# Autodesk Inventor assembly: Atom_3_Lite_Upgrade
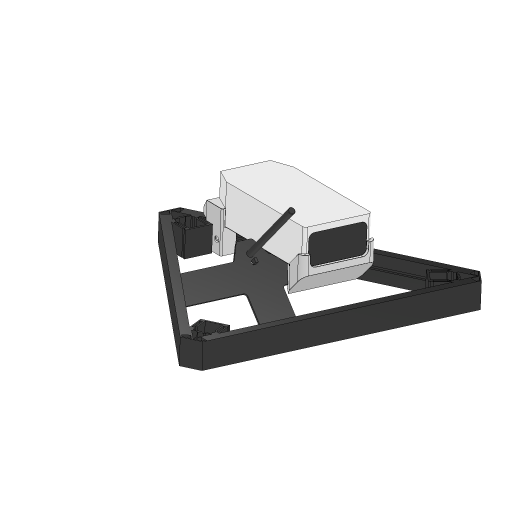
[picture p0: Inventor's stored thumbnail of the model, 512x512]
Saved by Autodesk Inventor 2024.3 (Build 283343000, 343)
## iProperties
Created: 2024-09-15
Part Number: Atom_3_Lite_Upgrade
Document SubType Name: Assembly
Designer: user
Author: user
## Documents named in this file (5)
- D:\Code\3D-Printing-Slicer-Settings\3D_Printer\Atom_3_Lite\[Machine_Upgrade]\Assembly\Atom_3_Lite_Upgrade.iam
- D:\Code\3D-Printing-Slicer-Settings\3D_Printer\Atom_3_Lite\[Machine_Upgrade]\Part\Atom_3_lite.ipt
- D:\Code\3D-Printing-Slicer-Settings\3D_Printer\Atom_3_Lite\[Machine_Upgrade]\Part\eBox.ipt
- D:\Code\3D-Printing-Slicer-Settings\3D_Printer\Atom_3_Lite\[Machine_Upgrade]\Part\esun_ebox_holder_front.ipt
- D:\Code\3D-Printing-Slicer-Settings\3D_Printer\Atom_3_Lite\[Machine_Upgrade]\Part\esun_ebox_holder_rear.ipt
## Components (4 placed, 4 different names)
1. Atom_3_lite:1 — 貼合:1, 相切:1, 相切:2, 貼合:2, 齊平:1, 貼合:4
2. eBox:1 — 貼合:1, 相切:1, 相切:2, 貼合:2, 貼合:3
3. esun_ebox_holder_front:1 — 貼合:3, 齊平:1, 貼合:4, 齊平:2, 齊平:3, 齊平:4, 齊平:5
4. esun_ebox_holder_rear:1 — 齊平:2, 齊平:3, 齊平:4, 齊平:5
## Relationships (11: Flush 5, Mate 4, Tangent 2)
- 貼合:1 [Mate]: Atom_3_lite:1 ↔ eBox:1
- 相切:1 [Tangent]: Atom_3_lite:1 ↔ eBox:1
- 相切:2 [Tangent]: Atom_3_lite:1 ↔ eBox:1
- 貼合:2 [Mate]: Atom_3_lite:1 ↔ eBox:1
- 貼合:3 [Mate]: eBox:1 ↔ esun_ebox_holder_front:1
- 齊平:1 [Flush]: Atom_3_lite:1 ↔ esun_ebox_holder_front:1
- 貼合:4 [Mate]: Atom_3_lite:1 ↔ esun_ebox_holder_front:1
- 齊平:2 [Flush]: esun_ebox_holder_front:1 ↔ esun_ebox_holder_rear:1
- 齊平:3 [Flush]: esun_ebox_holder_front:1 ↔ esun_ebox_holder_rear:1
- 齊平:4 [Flush]: esun_ebox_holder_front:1 ↔ esun_ebox_holder_rear:1
- 齊平:5 [Flush]: esun_ebox_holder_front:1 ↔ esun_ebox_holder_rear:1
